# Autodesk Inventor assembly: EL2-900
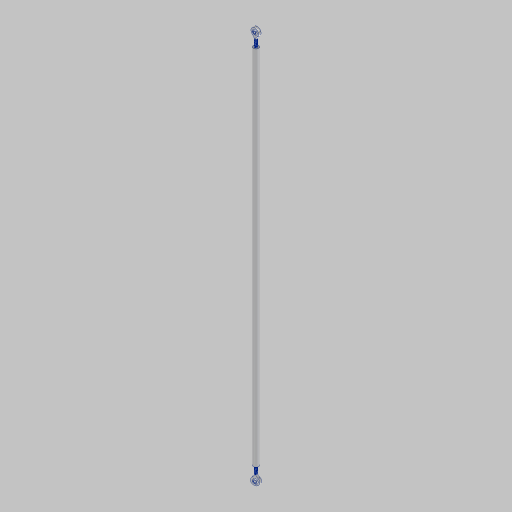
[picture p0: Inventor's stored thumbnail of the model, 512x512]
Saved by Autodesk Inventor 2023.5 (Build 275446000, 446)
## iProperties
Created: 2025-02-12
Part Number: EL2-900
Document SubType Name: Assembly
Designer: slick
Author: slick
## Documents named in this file (3)
- C:\Users\slick\OneDrive\Desktop\2025-ReefScape---CAD\Elevator\EL2\EL2-900.iam
- C:\Users\slick\OneDrive\Desktop\2025-ReefScape---CAD\Elevator\EL2\EL2-025.ipt
- C:\Users\slick\OneDrive\Desktop\2025-ReefScape---CAD\COMMON PARTS\MCMASTER\60645K812_Ball Joint Rod End\60645K812_Ball Joint Rod End.ipt
## Components (3 placed, 2 different names)
1. EL2-025:1 — Mate:1, Mate:2, Mate:3, Mate:4
2. 60645K812_Ball Joint Rod End:1 — Mate:1, Mate:4
3. 60645K812_Ball Joint Rod End:2 — Mate:2, Mate:3
## Relationships (4: Mate 4)
- Mate:1: EL2-025:1 ↔ 60645K812_Ball Joint Rod End:1
- Mate:2: EL2-025:1 ↔ 60645K812_Ball Joint Rod End:2
- Mate:3 (31.75 mm): EL2-025:1 ↔ 60645K812_Ball Joint Rod End:2
- Mate:4 (31.75 mm): EL2-025:1 ↔ 60645K812_Ball Joint Rod End:1
